# Autodesk Inventor assembly: Skateboard Remote
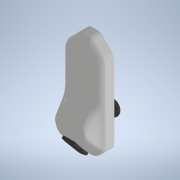
[picture p0: Inventor's stored thumbnail of the model, 180x180]
Saved by Autodesk Inventor 2020 (Build 240168000, 168)
## iProperties
Created: 2021-01-14
Part Number: Skateboard Remote
Document SubType Name: Assembly
Designer: Luke
Author: Luke
## Documents named in this file (16)
- C:\Users\Luke\Documents\Git Projects\Electric Skateboard V2\Part Files\Remote Parts\Skateboard Remote.iam
- C:\Users\Luke\Documents\Git Projects\Electric Skateboard V2\Part Files\Remote Parts\PCB.ipt
- C:\Users\Luke\Documents\Git Projects\Electric Skateboard V2\Part Files\Remote Parts\Battery Spacer.ipt
- C:\Users\Luke\Documents\Git Projects\Electric Skateboard V2\Part Files\Remote Parts\Battery.ipt
- C:\Users\Luke\Documents\Git Projects\Electric Skateboard V2\Part Files\Remote Parts\Button Module.ipt
- C:\Users\Luke\Documents\Git Projects\Electric Skateboard V2\Part Files\Remote Parts\Joystick.ipt
- C:\Users\Luke\Documents\Git Projects\Electric Skateboard V2\Part Files\Remote Parts\Button.ipt
- C:\Users\Luke\Documents\Git Projects\Electric Skateboard V2\Part Files\Remote Parts\Joystick Cap.ipt
- C:\Users\Luke\Documents\Git Projects\Electric Skateboard V2\Part Files\Remote Parts\Display.ipt
- C:\Users\Luke\Documents\Git Projects\Electric Skateboard V2\Part Files\Remote Parts\Vibrator Motor.ipt
- C:\Users\Luke\Documents\Git Projects\Electric Skateboard V2\Part Files\Remote Parts\USB Port.ipt
- C:\Users\Luke\Documents\Git Projects\Electric Skateboard V2\Part Files\Remote Parts\BMS.ipt
- C:\Users\Luke\Documents\Git Projects\Electric Skateboard V2\Part Files\Remote Parts\Button Holder Bottom Shifted Up More.ipt
- C:\Users\Luke\Documents\Git Projects\Electric Skateboard V2\Part Files\Remote Parts\Button Holder Top Shifted Up More.ipt
- C:\Users\Luke\Documents\Git Projects\Electric Skateboard V2\Part Files\Remote Parts\Finger Button.ipt
- C:\Users\Luke\Documents\Git Projects\Electric Skateboard V2\Part Files\Remote Parts\Enclosure Bottom Slim.ipt
## Components (18 placed, 15 different names)
1. PCB:1 — Mate:1, Flush:1, Flush:2, Mate:2, Flush:6, Flush:8, Flush:9, Flush:10, Flush:12, Mate:23, Mate:24, Mate:25, Mate:27, Mate:28, Mate:29, Mate:30, Flush:15, Mate:31, Mate:32, Flush:16, Mate:37, Mate:38, Mate:50, Flush:30, Flush:31, Mate:59, Flush:32
2. Battery Spacer:1 — Mate:1, Flush:1, Flush:2, Flush:3
3. Battery:1 — Flush:3, Mate:2, Flush:12
4. Button Module:1 — Mate:6, Mate:7, Mate:8, Mate:9, Mate:10, Mate:11, Mate:40, Mate:41, Flush:19
5. Joystick:1 — Flush:6, Flush:8, Flush:9, Flush:10, Mate:21, Mate:22, Mate:26
6. Button:3 — Mate:9, Mate:10, Mate:11, Mate:54, Mate:56, Mate:58
7. Button:2 — Mate:6, Mate:7, Mate:8, Mate:55, Flush:29, Mate:57
8. Joystick Cap:1 — Mate:21, Mate:22
9. Display:1 — Mate:23, Mate:24, Mate:25, Mate:26
10. Vibrator Motor:1 — Mate:27, Mate:28, Mate:29
11. USB Port:1 — Mate:30, Flush:15, Mate:31
12. BMS:1 — Mate:32, Flush:16, Mate:33, Flush:17, Mate:34, Flush:30
13. USB Port:2 — Mate:33, Flush:17, Mate:34
14. Button Holder Top Shifted Up More:1 — Mate:35, Mate:36, Mate:37, Mate:38, Mate:50, Flush:24
15. Button Holder Bottom Shifted Up More:1 — Mate:35, Mate:36, Mate:40, Mate:41, Flush:19, Flush:24
16. Finger Button:2 — Mate:54, Mate:56, Mate:58
17. Finger Button:1 — Mate:55, Flush:29, Mate:57
18. Enclosure Bottom Slim:1 — Flush:31, Mate:59, Flush:32
## Relationships (52: Mate 35, Flush 17)
- Mate:1: PCB:1 ↔ Battery Spacer:1
- Flush:1 (9.27 mm): PCB:1 ↔ Battery Spacer:1
- Flush:2 (6.4 mm): PCB:1 ↔ Battery Spacer:1
- Flush:3: Battery Spacer:1 ↔ Battery:1
- Mate:2: PCB:1 ↔ Battery:1
- Flush:6: PCB:1 ↔ Joystick:1
- Flush:8: PCB:1 ↔ Joystick:1
- Flush:9: PCB:1 ↔ Joystick:1
- Flush:10: PCB:1 ↔ Joystick:1
- Mate:6: Button Module:1 ↔ Button:2
- Mate:7: Button Module:1 ↔ Button:2
- Mate:8: Button Module:1 ↔ Button:2
- Mate:9: Button Module:1 ↔ Button:3
- Mate:10: Button Module:1 ↔ Button:3
- Mate:11: Button Module:1 ↔ Button:3
- Flush:12 (4 mm): PCB:1 ↔ Battery:1
- Mate:21: Joystick:1 ↔ Joystick Cap:1
- Mate:22: Joystick:1 ↔ Joystick Cap:1
- Mate:23: PCB:1 ↔ Display:1
- Mate:24: PCB:1 ↔ Display:1
- Mate:25: PCB:1 ↔ Display:1
- Mate:26 (5.5 mm): Joystick:1 ↔ Display:1
- Mate:27: PCB:1 ↔ Vibrator Motor:1
- Mate:28 (-12 mm): PCB:1 ↔ Vibrator Motor:1
- Mate:29 (-17 mm): PCB:1 ↔ Vibrator Motor:1
- Mate:30: PCB:1 ↔ USB Port:1
- Flush:15: PCB:1 ↔ USB Port:1
- Mate:31: PCB:1 ↔ USB Port:1
- Mate:32: PCB:1 ↔ BMS:1
- Flush:16: PCB:1 ↔ BMS:1
- Mate:33: BMS:1 ↔ USB Port:2
- Flush:17: BMS:1 ↔ USB Port:2
- Mate:34: BMS:1 ↔ USB Port:2
- Mate:35: Button Holder Top Shifted Up More:1 ↔ Button Holder Bottom Shifted Up More:1
- Mate:36: Button Holder Top Shifted Up More:1 ↔ Button Holder Bottom Shifted Up More:1
- Mate:37: PCB:1 ↔ Button Holder Top Shifted Up More:1
- Mate:38: PCB:1 ↔ Button Holder Top Shifted Up More:1
- Mate:40: Button Module:1 ↔ Button Holder Bottom Shifted Up More:1
- Mate:41: Button Module:1 ↔ Button Holder Bottom Shifted Up More:1
- Flush:19: Button Module:1 ↔ Button Holder Bottom Shifted Up More:1
- Mate:50: PCB:1 ↔ Button Holder Top Shifted Up More:1
- Flush:24: Button Holder Top Shifted Up More:1 ↔ Button Holder Bottom Shifted Up More:1
- Mate:54: Button:3 ↔ Finger Button:2
- Mate:55: Button:2 ↔ Finger Button:1
- Mate:56: Button:3 ↔ Finger Button:2
- Flush:29: Button:2 ↔ Finger Button:1
- Mate:57: Button:2 ↔ Finger Button:1
- Mate:58: Button:3 ↔ Finger Button:2
- Flush:30 (8.38 mm): PCB:1 ↔ BMS:1
- Flush:31: PCB:1 ↔ Enclosure Bottom Slim:1
- Mate:59: PCB:1 ↔ Enclosure Bottom Slim:1
- Flush:32: PCB:1 ↔ Enclosure Bottom Slim:1
